# Autodesk Inventor assembly: License plate in holder
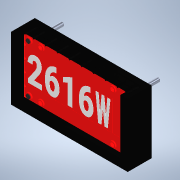
[picture p0: Inventor's stored thumbnail of the model, 180x180]
Saved by Autodesk Inventor 2022.2 (Build 262287010, 287A)
## iProperties
Created: 2022-06-18
Part Number: License plate in holder
Document SubType Name: Assembly
Designer: Main Account
Author: Main Account
## Documents named in this file (5)
- D:\Documents\Inventor\VEX\Custom Library\License plate in holder.iam
- D:\Documents\Inventor\VEX\Custom Library\License Plate Holder.ipt
- D:\Documents\Inventor\VEX\Custom Library\Double sided license plate.iam
- D:\Documents\Inventor\VEX\Library Backup\Library 1.3\Structure\Hardware\Screw Steel - Star\SScrew Star Smooth .875.ipt
- D:\Documents\Inventor\VEX\Library Backup\Library 1.3\Structure\Hardware\Screw Steel - Star.ipt
## Components (4 placed, 3 different names)
1. License Plate Holder:1 — Mate:1, Mate:2, Mate:3, Insert:1, Insert:2
2. Double sided license plate:2 [sub-assembly] — Mate:1, Mate:2, Mate:3
3. SScrew Star Smooth .875:1 — Insert:1
4. SScrew Star Smooth .875:2 — Insert:2
## Relationships (5: Mate 3, Insert 2)
- Mate:1: License Plate Holder:1 ↔ Double sided license plate:2
- Mate:2: License Plate Holder:1 ↔ Double sided license plate:2
- Mate:3 (0.15 mm): License Plate Holder:1 ↔ Double sided license plate:2
- Insert:1: License Plate Holder:1 ↔ SScrew Star Smooth .875:1
- Insert:2: License Plate Holder:1 ↔ SScrew Star Smooth .875:2
